# Autodesk Inventor assembly: lanceur-abeille
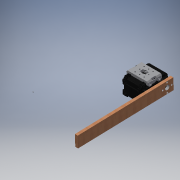
[picture p0: Inventor's stored thumbnail of the model, 180x180]
Saved by Autodesk Inventor 2017 (Build 210142000, 142)
## iProperties
Created: 2018-04-02
Part Number: lanceur-abeille
Document SubType Name: Assembly
Designer: franc
Author: franc
## Documents named in this file (4)
- C:\Users\franc\Desktop\EsialRobotik\Mecanique\2018\robot\abeille\lanceur-abeille.iam
- C:\Users\franc\Desktop\EsialRobotik\Mecanique\2018\robot\abeille\bras-lanceur.ipt
- C:\Users\franc\Desktop\EsialRobotik\Mecanique\composants\AX12\AX12.iam
- C:\Users\franc\Desktop\EsialRobotik\Mecanique\composants\AX12\F3.ipt
## Components (3 placed, 3 different names)
1. bras-lanceur:1 — Placage:1, Placage:2, Placage:3, Placage:4
2. AX12:1 [sub-assembly] — Placage:1, Placage:2, Placage:3, Placage:4, Placage:5, Placage:6, Placage:7
3. F3:1 — Placage:5, Placage:6, Placage:7
## Relationships (7: Mate 7)
- Placage:1 [Mate]: bras-lanceur:1 ↔ AX12:1
- Placage:2 [Mate]: bras-lanceur:1 ↔ AX12:1
- Placage:3 [Mate]: bras-lanceur:1 ↔ AX12:1
- Placage:4 [Mate]: bras-lanceur:1 ↔ AX12:1
- Placage:5 [Mate]: AX12:1 ↔ F3:1
- Placage:6 [Mate]: AX12:1 ↔ F3:1
- Placage:7 [Mate]: AX12:1 ↔ F3:1
